# Autodesk Inventor assembly: k2
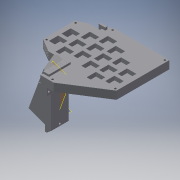
[picture p0: Inventor's stored thumbnail of the model, 180x180]
Saved by Autodesk Inventor 2017 (Build 210142000, 142)
## iProperties
Created: 2017-02-07
Part Number: k2
Document SubType Name: Assembly
Designer: herman
Author: herman
## Documents named in this file (10)
- C:\Users\herman\Documents\k2.iam
- C:\Users\herman\Documents\k2_l1.ipt
- C:\Users\herman\Documents\k2_l4.ipt
- C:\Users\herman\Documents\k2_l3.ipt
- C:\Users\herman\Documents\k2_l2.ipt
- C:\Users\herman\Documents\k2_t_leg.ipt
- C:\Users\herman\Documents\k2_t_l3.ipt
- C:\Users\herman\Documents\k2_t_l2.ipt
- C:\Users\herman\Documents\k2_t_l1a.ipt
- C:\Users\herman\Documents\k2_t_l4.ipt
## Components (9 placed, 9 different names)
1. k2_l4:1 — Mate:24, Mate:25
2. k2_l3:1 — Mate:1, Mate:6, Mate:24, Mate:25
3. k2_l1:1 — Mate:2, Mate:3, Mate:8, Mate:9, Mate:19, Mate:20
4. k2_l2:1 — Mate:1, Mate:2, Mate:3, Mate:6
5. k2_t_leg:1 — Mate:8, Mate:9
6. k2_t_l3:1 — Mate:14, Mate:15, Mate:21, Mate:22
7. k2_t_l2:1 — Mate:14, Mate:15, Mate:23, Mate:26
8. k2_t_l1a:1 — Mate:23, Mate:26
9. k2_t_l4:1 — Mate:19, Mate:20, Mate:21, Mate:22
## Relationships (16: Mate 16)
- Mate:1: k2_l3:1 ↔ k2_l2:1
- Mate:2: k2_l1:1 ↔ k2_l2:1
- Mate:3: k2_l1:1 ↔ k2_l2:1
- Mate:6: k2_l3:1 ↔ k2_l2:1
- Mate:8: k2_l1:1 ↔ k2_t_leg:1
- Mate:9: k2_l1:1 ↔ k2_t_leg:1
- Mate:14: k2_t_l3:1 ↔ k2_t_l2:1
- Mate:15: k2_t_l3:1 ↔ k2_t_l2:1
- Mate:19: k2_l1:1 ↔ k2_t_l4:1
- Mate:20: k2_l1:1 ↔ k2_t_l4:1
- Mate:21: k2_t_l3:1 ↔ k2_t_l4:1
- Mate:22: k2_t_l3:1 ↔ k2_t_l4:1
- Mate:23: k2_t_l2:1 ↔ k2_t_l1a:1
- Mate:24: k2_l4:1 ↔ k2_l3:1
- Mate:25: k2_l4:1 ↔ k2_l3:1
- Mate:26: k2_t_l2:1 ↔ k2_t_l1a:1
